# Autodesk Inventor assembly: Ciąg
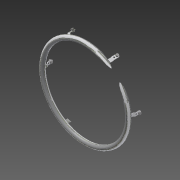
[picture p0: Inventor's stored thumbnail of the model, 180x180]
Saved by Autodesk Inventor 2015 (Build 190159000, 159)
## iProperties
Created: 2016-01-12
Part Number: Ciąg
Document SubType Name: Konstrukcja spawana
Designer: graaapsik
Weld Material: Aluminium 6061-AHC
Author: graaapsik
## Documents named in this file (5)
- C:\Users\EriveltonDell\Documents\Centro Universitário da FEI\Wheelchair\CADEIRA DE RODAS - DESENHO\Model\Ciąg.iam
- C:\Users\EriveltonDell\Documents\Centro Universitário da FEI\Wheelchair\CADEIRA DE RODAS - DESENHO\Model\Ciąg.ipt
- C:\Users\EriveltonDell\Documents\Centro Universitário da FEI\Wheelchair\CADEIRA DE RODAS - DESENHO\Model\Blaszka_do_ciągu.ipt
- C:\Users\EriveltonDell\Documents\Centro Universitário da FEI\Wheelchair\CADEIRA DE RODAS - DESENHO\Model\ISO 1207 - M10 x 12.ipt
- C:\Users\EriveltonDell\Documents\Centro Universitário da FEI\Wheelchair\CADEIRA DE RODAS - DESENHO\Model\ISO 4032 - M10ISO.ipt
## Components (19 placed, 4 different names)
1. Ciąg:1 — Równoległy:3
2. Blaszka_do_ciągu:1 — Zestawiający:26, Równoległy:2, Równoległy:3, Wstaw:1
3. Blaszka_do_ciągu:7
4. Blaszka_do_ciągu:8
5. Blaszka_do_ciągu:9
6. Blaszka_do_ciągu:10
7. Blaszka_do_ciągu:11
8. ISO 1207 M10 x 12:1 — Zestawiający:27, Wstaw:1, Wstaw:2
9. ISO 4032 M10:1 — Zestawiający:27, Wstaw:2
10. ISO 1207 M10 x 12:2
11. ISO 4032 M10:2
12. ISO 1207 M10 x 12:3
13. ISO 4032 M10:3
14. ISO 1207 M10 x 12:4
15. ISO 4032 M10:4
16. ISO 1207 M10 x 12:5
17. ISO 4032 M10:5
18. ISO 1207 M10 x 12:6
19. ISO 4032 M10:6
## Component patterns: (6 elements, first: Blaszka_do_ciągu:1), (6 elements, first: ISO 1207 M10 x 12:1 + ISO 4032 M10:1)
## Relationships (6: Mate 2, Flush 2, Insert 2)
- Zestawiający:26 [Mate] (-10 mm): Blaszka_do_ciągu:1
- Równoległy:2 [Flush] (-251.25 mm): Blaszka_do_ciągu:1
- Równoległy:3 [Flush] (15 mm): Ciąg:1 ↔ Blaszka_do_ciągu:1
- Zestawiający:27 [Mate]: ISO 1207 M10 x 12:1 ↔ ISO 4032 M10:1
- Wstaw:1 [Insert]: Blaszka_do_ciągu:1 ↔ ISO 1207 M10 x 12:1
- Wstaw:2 [Insert] (2 mm): ISO 1207 M10 x 12:1 ↔ ISO 4032 M10:1
